# Autodesk Inventor assembly: HOUSING
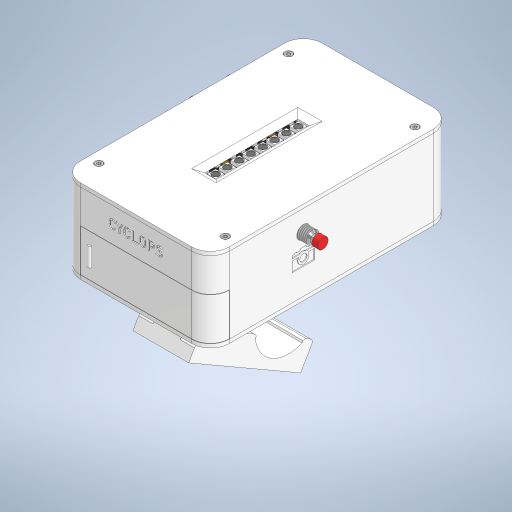
[picture p0: Inventor's stored thumbnail of the model, 512x512]
Saved by Autodesk Inventor 2023 (Build 270158000, 158)
## iProperties
Created: 2023-03-14
Part Number: HOUSING
Document SubType Name: Assembly
Designer: Amos Yu
Author: Amos Yu
## Documents named in this file (17)
- C:\Users\Dell\Documents\capstone\cyclops\src\cad\front_housing\HOUSING.iam
- C:\Users\Dell\Documents\capstone\cyclops\src\cad\front_housing\BOTTOM.ipt
- C:\Users\Dell\Documents\capstone\cyclops\src\cad\front_housing\TOP.ipt
- C:\Users\Dell\Documents\capstone\cyclops\src\cad\front_housing\MIDDLE.ipt
- C:\Users\Dell\Documents\capstone\cyclops\src\cad\BOLT.ipt
- C:\Users\Dell\Documents\capstone\cyclops\src\cad\NUT.ipt
- C:\Users\Dell\Documents\capstone\cyclops\src\cad\RASPBERRY PI.ipt
- C:\Users\Dell\Documents\capstone\cyclops\src\cad\BUTTON.ipt
- C:\Users\Dell\Documents\capstone\cyclops\src\cad\CAMERA.ipt
- C:\Users\Dell\Documents\capstone\cyclops\src\cad\bike_mount\BIKE_MOUNT_BOTTOM.ipt
- C:\Users\Dell\Documents\capstone\cyclops\src\cad\bike_mount\BIKE_MOUNT_TOP.ipt
- C:\Users\Dell\Documents\capstone\cyclops\src\cad\ACCELEROMETER.ipt
- C:\Users\Dell\Documents\capstone\cyclops\src\cad\front_housing\DOOR.ipt
- C:\Users\Dell\Documents\capstone\cyclops\src\cad\front_housing\PARAMETERS.ipt
- C:\Users\Dell\Documents\capstone\cyclops\src\cad\LED.ipt
- C:\Users\Dell\Documents\capstone\cyclops\src\cad\front_housing\WIRE_HOUSING.ipt
- C:\Users\Dell\Documents\capstone\cyclops\src\cad\front_housing\LED_HOUSING.ipt
## Components (47 placed, 15 different names)
1. BOTTOM:1 — Flush:1, Flush:2, Flush:3, Mate:1, Flush:4, Flush:5, Mate:3, Mate:4, Mate:5, Mate:6, Mate:7, Mate:8, Mate:9, Mate:10, Mate:36, Mate:37, Mate:38, Mate:43, Mate:44, Mate:45, Mate:46, Mate:47, Mate:48, Mate:49, Mate:50, Mate:57, Mate:58, Mate:59, Mate:60, Mate:68, Mate:70, Mate:86
2. TOP:1 — Flush:6, Flush:7, Mate:2, Mate:23, Mate:24, Mate:25, Mate:26, Mate:28, Mate:29, Mate:30, Mate:31, Mate:75, Mate:76, Mate:77, Mate:80, Mate:81, Mate:96, Mate:98, Mate:106, Mate:107, Mate:112
3. MIDDLE:1 — Mate:1, Flush:4, Flush:5, Flush:6, Flush:7, Mate:2, Mate:61, Mate:62, Mate:63, Mate:64, Mate:65, Mate:66, Mate:67, Mate:87, Angle:8, Mate:88, Angle:9, Mate:89, Angle:10, Mate:90, Angle:11, Mate:91, Angle:12, Mate:92, Angle:13, Mate:93, Angle:14, Mate:94, Angle:15, Mate:95
4. DOOR:1 — Mate:86, Flush:9, Mate:87
5. WIRE_HOUSING:1 — Mate:101, Mate:102, Mate:103, Mate:104, Mate:105
6. BIKE_MOUNT_BOTTOM:1 — Mate:69, Flush:8, Angle:5
7. BIKE_MOUNT_TOP:1 — Mate:69, Flush:8, Mate:70, Mate:71, Mate:72, Angle:6, Angle:7, Mate:73, Mate:74
8. RASPBERRY PI:1 — Mate:36, Mate:37, Mate:38, Mate:53, Mate:54, Mate:101, Mate:102, Mate:103
9. CAMERA:1 — Mate:67, Angle:4, Mate:68
10. BUTTON:1 — Mate:63, Mate:66, Angle:3
11. BUTTON:2 — Mate:62, Mate:65, Angle:2
12. BUTTON:3 — Mate:61, Mate:64, Angle:1
13. ACCELEROMETER:1 — Mate:75, Mate:76, Mate:77, Mate:97, Mate:99
14. LED:1 — Mate:109, Mate:110, Mate:112
15. LED_HOUSING:1 — Mate:106, Mate:107, Mate:109, Mate:110, Mate:111
16. BOLT:1 — Mate:3, Mate:7, Mate:13
17. NUT:1 — Mate:11, Angle:9, Mate:89
18. BOLT:2 — Mate:4, Mate:8, Mate:11
19. NUT:2 — Mate:12, Angle:14, Mate:94
20. BOLT:3 — Mate:5, Mate:10, Mate:12
21. NUT:3 — Mate:13, Angle:11, Mate:91
22. BOLT:4 — Mate:6, Mate:9, Mate:14
23. NUT:4 — Mate:14, Angle:12, Mate:92
24. BOLT:5 — Mate:23, Mate:27, Mate:28
25. NUT:5 — Mate:27, Angle:15, Mate:95
26. BOLT:6 — Mate:16, Mate:24, Mate:31
27. NUT:6 — Mate:16, Angle:13, Mate:93
28. BOLT:7 — Mate:17, Mate:25, Mate:30
29. NUT:7 — Mate:17, Angle:10, Mate:90
30. BOLT:8 — Mate:18, Mate:26, Mate:29
31. NUT:8 — Mate:18, Angle:8, Mate:88
32. BOLT:9 — Mate:39, Mate:43, Mate:47
33. NUT:9 — Mate:39, Mate:53
34. BOLT:10 — Mate:40, Mate:46, Mate:49
35. NUT:10 — Mate:40, Mate:105
36. BOLT:11 — Mate:41, Mate:45, Mate:48
37. NUT:11 — Mate:41, Mate:104
38. BOLT:12 — Mate:42, Mate:44, Mate:50
39. NUT:12 — Mate:42, Mate:54
40. BOLT:13 — Mate:55, Mate:58, Mate:60, Mate:71
41. NUT:13 — Mate:55, Angle:7, Mate:74
42. BOLT:14 — Mate:56, Mate:57, Mate:59, Mate:72
43. NUT:14 — Mate:56, Angle:6, Mate:73
44. BOLT:15 — Mate:78, Mate:81, Mate:96
45. NUT:15 — Mate:78, Mate:97
46. BOLT:16 — Mate:79, Mate:80, Mate:98, Mate:111
47. NUT:16 — Mate:79, Mate:99
## Relationships (119: Mate 95, Angle 15, Flush 9)
- Flush:1: BOTTOM:1
- Flush:2: BOTTOM:1
- Flush:3: BOTTOM:1
- Mate:1: BOTTOM:1 ↔ MIDDLE:1
- Flush:4: BOTTOM:1 ↔ MIDDLE:1
- Flush:5: BOTTOM:1 ↔ MIDDLE:1
- Flush:6: TOP:1 ↔ MIDDLE:1
- Flush:7: TOP:1 ↔ MIDDLE:1
- Mate:2: TOP:1 ↔ MIDDLE:1
- Mate:3: BOTTOM:1 ↔ BOLT:1
- Mate:4: BOTTOM:1 ↔ BOLT:2
- Mate:5: BOTTOM:1 ↔ BOLT:3
- Mate:6: BOTTOM:1 ↔ BOLT:4
- Mate:7: BOTTOM:1 ↔ BOLT:1
- Mate:8: BOTTOM:1 ↔ BOLT:2
- Mate:9: BOTTOM:1 ↔ BOLT:4
- Mate:10: BOTTOM:1 ↔ BOLT:3
- Mate:11: NUT:1 ↔ BOLT:2
- Mate:12: NUT:2 ↔ BOLT:3
- Mate:13: BOLT:1 ↔ NUT:3
- Mate:14: BOLT:4 ↔ NUT:4
- Mate:16: BOLT:6 ↔ NUT:6
- Mate:17: BOLT:7 ↔ NUT:7
- Mate:18: BOLT:8 ↔ NUT:8
- Mate:23: TOP:1 ↔ BOLT:5
- Mate:24: TOP:1 ↔ BOLT:6
- Mate:25: TOP:1 ↔ BOLT:7
- Mate:26: TOP:1 ↔ BOLT:8
- Mate:27: BOLT:5 ↔ NUT:5
- Mate:28: TOP:1 ↔ BOLT:5
- Mate:29: TOP:1 ↔ BOLT:8
- Mate:30: TOP:1 ↔ BOLT:7
- Mate:31: TOP:1 ↔ BOLT:6
- Mate:36: BOTTOM:1 ↔ RASPBERRY PI:1
- Mate:37: BOTTOM:1 ↔ RASPBERRY PI:1
- Mate:38: BOTTOM:1 ↔ RASPBERRY PI:1
- Mate:39: BOLT:9 ↔ NUT:9
- Mate:40: BOLT:10 ↔ NUT:10
- Mate:41: BOLT:11 ↔ NUT:11
- Mate:42: BOLT:12 ↔ NUT:12
- Mate:43: BOTTOM:1 ↔ BOLT:9
- Mate:44: BOTTOM:1 ↔ BOLT:12
- Mate:45: BOTTOM:1 ↔ BOLT:11
- Mate:46: BOTTOM:1 ↔ BOLT:10
- Mate:47: BOTTOM:1 ↔ BOLT:9
- Mate:48: BOTTOM:1 ↔ BOLT:11
- Mate:49: BOTTOM:1 ↔ BOLT:10
- Mate:50: BOTTOM:1 ↔ BOLT:12
- Mate:53: RASPBERRY PI:1 ↔ NUT:9
- Mate:54: RASPBERRY PI:1 ↔ NUT:12
- Mate:55: BOLT:13 ↔ NUT:13
- Mate:56: BOLT:14 ↔ NUT:14
- Mate:57: BOTTOM:1 ↔ BOLT:14
- Mate:58: BOTTOM:1 ↔ BOLT:13
- Mate:59: BOTTOM:1 ↔ BOLT:14
- Mate:60: BOTTOM:1 ↔ BOLT:13
- Mate:61: MIDDLE:1 ↔ BUTTON:3
- Mate:62: MIDDLE:1 ↔ BUTTON:2
- Mate:63: MIDDLE:1 ↔ BUTTON:1
- Mate:64: MIDDLE:1 ↔ BUTTON:3
- Mate:65: MIDDLE:1 ↔ BUTTON:2
- Mate:66: MIDDLE:1 ↔ BUTTON:1
- Angle:1 (0 deg): BUTTON:3
- Angle:2 (0 deg): BUTTON:2
- Angle:3 (0 deg): BUTTON:1
- Mate:67: MIDDLE:1 ↔ CAMERA:1
- Angle:4 (180 deg): CAMERA:1
- Mate:68: BOTTOM:1 ↔ CAMERA:1
- Mate:69: BIKE_MOUNT_BOTTOM:1 ↔ BIKE_MOUNT_TOP:1
- Flush:8: BIKE_MOUNT_BOTTOM:1 ↔ BIKE_MOUNT_TOP:1
- Mate:70: BOTTOM:1 ↔ BIKE_MOUNT_TOP:1
- Mate:71: BIKE_MOUNT_TOP:1 ↔ BOLT:13
- Mate:72: BIKE_MOUNT_TOP:1 ↔ BOLT:14
- Angle:5 (150 deg): BIKE_MOUNT_BOTTOM:1
- Angle:6 (0 deg): BIKE_MOUNT_TOP:1 ↔ NUT:14
- Angle:7 (0 deg): BIKE_MOUNT_TOP:1 ↔ NUT:13
- Mate:73: BIKE_MOUNT_TOP:1 ↔ NUT:14
- Mate:74: BIKE_MOUNT_TOP:1 ↔ NUT:13
- Mate:75: TOP:1 ↔ ACCELEROMETER:1
- Mate:76: TOP:1 ↔ ACCELEROMETER:1
- Mate:77: TOP:1 ↔ ACCELEROMETER:1
- Mate:78: BOLT:15 ↔ NUT:15
- Mate:79: BOLT:16 ↔ NUT:16
- Mate:80: TOP:1 ↔ BOLT:16
- Mate:81: TOP:1 ↔ BOLT:15
- Mate:86 (0.2 mm): BOTTOM:1 ↔ DOOR:1
- Flush:9: DOOR:1
- Mate:87 (0.2 mm): MIDDLE:1 ↔ DOOR:1
- Angle:8 (0 deg): MIDDLE:1 ↔ NUT:8
- Mate:88: MIDDLE:1 ↔ NUT:8
- Angle:9 (0 deg): MIDDLE:1 ↔ NUT:1
- Mate:89: MIDDLE:1 ↔ NUT:1
- Angle:10 (0 deg): MIDDLE:1 ↔ NUT:7
- Mate:90: MIDDLE:1 ↔ NUT:7
- Angle:11 (0 deg): MIDDLE:1 ↔ NUT:3
- Mate:91: MIDDLE:1 ↔ NUT:3
- Angle:12 (0 deg): MIDDLE:1 ↔ NUT:4
- Mate:92: MIDDLE:1 ↔ NUT:4
- Angle:13 (0 deg): MIDDLE:1 ↔ NUT:6
- Mate:93: MIDDLE:1 ↔ NUT:6
- Angle:14 (0 deg): MIDDLE:1 ↔ NUT:2
- Mate:94: MIDDLE:1 ↔ NUT:2
- Angle:15 (0 deg): MIDDLE:1 ↔ NUT:5
- Mate:95: MIDDLE:1 ↔ NUT:5
- Mate:96: TOP:1 ↔ BOLT:15
- Mate:97: ACCELEROMETER:1 ↔ NUT:15
- Mate:98: TOP:1 ↔ BOLT:16
- Mate:99: ACCELEROMETER:1 ↔ NUT:16
- Mate:101: WIRE_HOUSING:1 ↔ RASPBERRY PI:1
- Mate:102: WIRE_HOUSING:1 ↔ RASPBERRY PI:1
- Mate:103: WIRE_HOUSING:1 ↔ RASPBERRY PI:1
- Mate:104: WIRE_HOUSING:1 ↔ NUT:11
- Mate:105: WIRE_HOUSING:1 ↔ NUT:10
- Mate:106: TOP:1 ↔ LED_HOUSING:1
- Mate:107: TOP:1 ↔ LED_HOUSING:1
- Mate:109: LED:1 ↔ LED_HOUSING:1
- Mate:110: LED:1 ↔ LED_HOUSING:1
- Mate:111: LED_HOUSING:1 ↔ BOLT:16
- Mate:112 (0.1 mm): TOP:1 ↔ LED:1
## Named parameters: total_depth = 130 mm, total_width = 80 mm, total_height = 45 mm, thickness = 2 mm, tol = 0.1 mm, fillet_outer_radius = 10 mm, lip_height = 5 mm, bolt_thread_diameter = 2 mm, bolt_head_diameter = 4 mm, bolt_inset_width = 6 mm, bolt_head_height = 2 mm, bolt_inset_depth = 14 mm, door_height = 23 mm
